# Autodesk Inventor assembly: Raspberry_Workbench
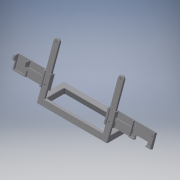
[picture p0: Inventor's stored thumbnail of the model, 180x180]
Saved by Autodesk Inventor 2017 (Build 210142000, 142)
## iProperties
Created: 2019-10-01
Part Number: Raspberry_Workbench
Document SubType Name: Assembly
Designer: Bear
Author: Bear
## Documents named in this file (5)
- E:\Work\Repos\personal\3d-design\02_Designs\02_work\rpi_support\rpi_support.iam
- E:\Work\Repos\personal\3d-design\02_Designs\02_work\rpi_support\rpi_support.ipt
- E:\Work\Repos\personal\3d-design\02_Designs\02_work\rpi_support\rpi_support_item_rfid.ipt
- E:\Work\Repos\personal\3d-design\02_Designs\02_work\rpi_support\rpi_support_item_fingerprint.ipt
- E:\Work\Repos\personal\3d-design\02_Designs\02_work\rpi_support\rpi_support.xlsx
## Components (3 placed, 3 different names)
1. rpi_support:1 — Mate:1, Mate:2, Mate:3, Mate:4
2. rpi_support_item_rfid:1 — Mate:1, Mate:2
3. rpi_support_item_fingerprint:1 — Mate:3, Mate:4
## Relationships (4: Mate 4)
- Mate:1 (0.1 mm): rpi_support:1 ↔ rpi_support_item_rfid:1
- Mate:2 (0.1 mm): rpi_support:1 ↔ rpi_support_item_rfid:1
- Mate:3 (0.1 mm): rpi_support:1 ↔ rpi_support_item_fingerprint:1
- Mate:4 (0.1 mm): rpi_support:1 ↔ rpi_support_item_fingerprint:1
## Named parameters: clearance = 0.1 mm, arm_angle = 70 deg, hole_diam = 3.1 mm, hole_h_space = 126.2 mm, hole_v_space = 65.65 mm, hole_b_space = 30 mm, arm_width = 12 mm, arm_thick = 4 mm, arm_rib_space = 1.25 mm, arm_rib_thick = 2 mm, base_width = 53 mm, base_thick = 10 mm, base_lenght = 138.2 mm, general_fillet = 1.5 mm, hole_to_border = 38 mm, hook_width = 25 mm, hook_thick = 2 mm, rfid_width = 39.5 mm, rfid_pin_border = 8 mm, rfid_pin_width = 5 mm, rfid_screw_diam = 3.1 mm, rfid_screw_h = 2.5 mm, rfid_screw_v = 15.5 mm, rfid_clock_pad = 3 mm, rfid_clock_h = 4.5 mm, rfid_clock_v = 8.5 mm, rfid_clock_thick = 1.5 mm, finger_width = 21 mm, finger_claw_h = 8 mm, finger_claw_pad = 14 mm, finger_claw_clip = 2 mm, finger_claw_v = 7.3 mm, finger_claw_ramp = 1 mm
